# Autodesk Inventor assembly: pitch_motor_flashlight_attached_model
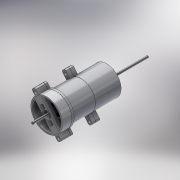
[picture p0: Inventor's stored thumbnail of the model, 180x180]
Saved by Autodesk Inventor 2018 (Build 220112000, 112)
## iProperties
Created: 2018-02-06
Part Number: pitch_motor_flashlight_attached_model
Document SubType Name: Assembly
Designer: mansu
Author: mansu
Sending System: SolidWorks 2017
Last Author: leoli
Last Saved: 2018-03-26
## Documents named in this file (7)
- F:\OneDrive\Documents\2018 UBC\ELEC 391\Motor\SolidWorks\Pitch\pitch_motor_flashlight_attached_model.iam
- F:\OneDrive\Documents\2018 UBC\ELEC 391\Motor\SolidWorks\Pitch\pitch_RotorCore.ipt
- F:\OneDrive\Documents\2018 UBC\ELEC 391\Motor\SolidWorks\Pitch\pitch_shaft.ipt
- F:\OneDrive\Documents\2018 UBC\ELEC 391\Motor\SolidWorks\Pitch\pitch_StatorShell_v5.ipt
- F:\OneDrive\Documents\2018 UBC\ELEC 391\Motor\SolidWorks\Pitch\pitch_StatorShell_v1_Top_Flashlight_attachment.ipt
- F:\OneDrive\Documents\2018 UBC\ELEC 391\Motor\SolidWorks\Pitch\pitch_commutator_attachment1.ipt
- F:\OneDrive\Documents\2018 UBC\ELEC 391\Motor\SolidWorks\Pitch\pitch_stator_front_attachment_flashlight.ipt
## Components (6 placed, 6 different names)
1. pitch_RotorCore:1 — Mate:2, Mate:6
2. pitch_shaft:1 — Mate:1, Mate:2, Mate:3, Mate:4, Mate:5
3. pitch_StatorShell_v5:1 — Mate:1, Mate:6, Mate:7, Mate:8
4. pitch_StatorShell_v1_Top_Flashlight_attachment:1 — Mate:4, Mate:9, Mate:10
5. pitch_commutator_attachment1:1 — Mate:5, Flush:1
6. pitch_stator_front_attachment_flashlight:1 — Mate:3, Mate:7, Mate:8, Flush:1, Mate:9, Mate:10
## Relationships (11: Mate 10, Flush 1)
- Mate:1: pitch_shaft:1 ↔ pitch_StatorShell_v5:1
- Mate:2: pitch_RotorCore:1 ↔ pitch_shaft:1
- Mate:3: pitch_shaft:1 ↔ pitch_stator_front_attachment_flashlight:1
- Mate:4: pitch_shaft:1 ↔ pitch_StatorShell_v1_Top_Flashlight_attachment:1
- Mate:5: pitch_shaft:1 ↔ pitch_commutator_attachment1:1
- Mate:6 (6 mm): pitch_RotorCore:1 ↔ pitch_StatorShell_v5:1
- Mate:7 (0.1 mm): pitch_StatorShell_v5:1 ↔ pitch_stator_front_attachment_flashlight:1
- Mate:8: pitch_StatorShell_v5:1 ↔ pitch_stator_front_attachment_flashlight:1
- Flush:1 (1 mm): pitch_commutator_attachment1:1 ↔ pitch_stator_front_attachment_flashlight:1
- Mate:9: pitch_StatorShell_v1_Top_Flashlight_attachment:1 ↔ pitch_stator_front_attachment_flashlight:1
- Mate:10 (0.1 mm): pitch_StatorShell_v1_Top_Flashlight_attachment:1 ↔ pitch_stator_front_attachment_flashlight:1
